(part 1 of 2)
# Autodesk Inventor assembly: Zynq_Z010_uZed_F_Prod
Saved by Autodesk Inventor 2015 (Build 190159000, 159)
## iProperties
Created: 2015-04-03
Part Number: Zynq_Z010_uZed_F_Prod
Document SubType Name: Assembly
Designer: -
Author: -
Author: Author
Title: Open CASCADE Shape Model
Organization: Open CASCADE
Description: Open CASCADE Model
Authority: Unknown
Creation Date: 2013-12-20
Sending System: Open CASCADE 6.2
Preprocessor: Open CASCADE STEP processor 6.2
## Documents named in this file (361)
- C:\Users\spichelh\Documents\GitHub\beta-hardware\Enclosure\Version 002\Imported Components\Zynq_Z010_uZed_F_Prod\Zynq_Z010_uZed_F_Prod.iam
- C:\Users\spichelh\Documents\GitHub\beta-hardware\Enclosure\Version 002\Imported Components\Zynq_Z010_uZed_F_Prod\Board.ipt
- C:\Users\spichelh\Documents\GitHub\beta-hardware\Enclosure\Version 002\Imported Components\Zynq_Z010_uZed_F_Prod\R96.iam
- C:\Users\spichelh\Documents\GitHub\beta-hardware\Enclosure\Version 002\Imported Components\Zynq_Z010_uZed_F_Prod\C220.iam
- C:\Users\spichelh\Documents\GitHub\beta-hardware\Enclosure\Version 002\Imported Components\Zynq_Z010_uZed_F_Prod\C219.iam
- C:\Users\spichelh\Documents\GitHub\beta-hardware\Enclosure\Version 002\Imported Components\Zynq_Z010_uZed_F_Prod\R91.iam
- C:\Users\spichelh\Documents\GitHub\beta-hardware\Enclosure\Version 002\Imported Components\Zynq_Z010_uZed_F_Prod\R90.iam
- C:\Users\spichelh\Documents\GitHub\beta-hardware\Enclosure\Version 002\Imported Components\Zynq_Z010_uZed_F_Prod\R89.iam
- C:\Users\spichelh\Documents\GitHub\beta-hardware\Enclosure\Version 002\Imported Components\Zynq_Z010_uZed_F_Prod\R88.iam
- C:\Users\spichelh\Documents\GitHub\beta-hardware\Enclosure\Version 002\Imported Components\Zynq_Z010_uZed_F_Prod\D1.iam
- C:\Users\spichelh\Documents\GitHub\beta-hardware\Enclosure\Version 002\Imported Components\Zynq_Z010_uZed_F_Prod\MTG3.iam
- C:\Users\spichelh\Documents\GitHub\beta-hardware\Enclosure\Version 002\Imported Components\Zynq_Z010_uZed_F_Prod\MTG4.iam
- C:\Users\spichelh\Documents\GitHub\beta-hardware\Enclosure\Version 002\Imported Components\Zynq_Z010_uZed_F_Prod\U11.iam
- C:\Users\spichelh\Documents\GitHub\beta-hardware\Enclosure\Version 002\Imported Components\Zynq_Z010_uZed_F_Prod\U5.iam
- C:\Users\spichelh\Documents\GitHub\beta-hardware\Enclosure\Version 002\Imported Components\Zynq_Z010_uZed_F_Prod\U6.iam
- C:\Users\spichelh\Documents\GitHub\beta-hardware\Enclosure\Version 002\Imported Components\Zynq_Z010_uZed_F_Prod\U10.iam
- C:\Users\spichelh\Documents\GitHub\beta-hardware\Enclosure\Version 002\Imported Components\Zynq_Z010_uZed_F_Prod\U13.iam
- C:\Users\spichelh\Documents\GitHub\beta-hardware\Enclosure\Version 002\Imported Components\Zynq_Z010_uZed_F_Prod\C41.iam
- C:\Users\spichelh\Documents\GitHub\beta-hardware\Enclosure\Version 002\Imported Components\Zynq_Z010_uZed_F_Prod\C170.iam
- C:\Users\spichelh\Documents\GitHub\beta-hardware\Enclosure\Version 002\Imported Components\Zynq_Z010_uZed_F_Prod\C176.iam
- C:\Users\spichelh\Documents\GitHub\beta-hardware\Enclosure\Version 002\Imported Components\Zynq_Z010_uZed_F_Prod\C181.iam
- C:\Users\spichelh\Documents\GitHub\beta-hardware\Enclosure\Version 002\Imported Components\Zynq_Z010_uZed_F_Prod\C188.iam
- C:\Users\spichelh\Documents\GitHub\beta-hardware\Enclosure\Version 002\Imported Components\Zynq_Z010_uZed_F_Prod\C42.iam
- C:\Users\spichelh\Documents\GitHub\beta-hardware\Enclosure\Version 002\Imported Components\Zynq_Z010_uZed_F_Prod\C190.iam
- C:\Users\spichelh\Documents\GitHub\beta-hardware\Enclosure\Version 002\Imported Components\Zynq_Z010_uZed_F_Prod\C179.iam
- C:\Users\spichelh\Documents\GitHub\beta-hardware\Enclosure\Version 002\Imported Components\Zynq_Z010_uZed_F_Prod\C189.iam
- C:\Users\spichelh\Documents\GitHub\beta-hardware\Enclosure\Version 002\Imported Components\Zynq_Z010_uZed_F_Prod\C169.iam
- C:\Users\spichelh\Documents\GitHub\beta-hardware\Enclosure\Version 002\Imported Components\Zynq_Z010_uZed_F_Prod\C193.iam
- C:\Users\spichelh\Documents\GitHub\beta-hardware\Enclosure\Version 002\Imported Components\Zynq_Z010_uZed_F_Prod\C196.iam
- C:\Users\spichelh\Documents\GitHub\beta-hardware\Enclosure\Version 002\Imported Components\Zynq_Z010_uZed_F_Prod\C200.iam
- C:\Users\spichelh\Documents\GitHub\beta-hardware\Enclosure\Version 002\Imported Components\Zynq_Z010_uZed_F_Prod\C203.iam
- C:\Users\spichelh\Documents\GitHub\beta-hardware\Enclosure\Version 002\Imported Components\Zynq_Z010_uZed_F_Prod\C173.iam
- C:\Users\spichelh\Documents\GitHub\beta-hardware\Enclosure\Version 002\Imported Components\Zynq_Z010_uZed_F_Prod\C175.iam
- C:\Users\spichelh\Documents\GitHub\beta-hardware\Enclosure\Version 002\Imported Components\Zynq_Z010_uZed_F_Prod\C171.iam
- C:\Users\spichelh\Documents\GitHub\beta-hardware\Enclosure\Version 002\Imported Components\Zynq_Z010_uZed_F_Prod\C183.iam
- C:\Users\spichelh\Documents\GitHub\beta-hardware\Enclosure\Version 002\Imported Components\Zynq_Z010_uZed_F_Prod\C43.iam
- C:\Users\spichelh\Documents\GitHub\beta-hardware\Enclosure\Version 002\Imported Components\Zynq_Z010_uZed_F_Prod\C199.iam
- C:\Users\spichelh\Documents\GitHub\beta-hardware\Enclosure\Version 002\Imported Components\Zynq_Z010_uZed_F_Prod\C194.iam
- C:\Users\spichelh\Documents\GitHub\beta-hardware\Enclosure\Version 002\Imported Components\Zynq_Z010_uZed_F_Prod\C186.iam
- C:\Users\spichelh\Documents\GitHub\beta-hardware\Enclosure\Version 002\Imported Components\Zynq_Z010_uZed_F_Prod\C184.iam
- C:\Users\spichelh\Documents\GitHub\beta-hardware\Enclosure\Version 002\Imported Components\Zynq_Z010_uZed_F_Prod\C44.iam
- C:\Users\spichelh\Documents\GitHub\beta-hardware\Enclosure\Version 002\Imported Components\Zynq_Z010_uZed_F_Prod\C202.iam
- C:\Users\spichelh\Documents\GitHub\beta-hardware\Enclosure\Version 002\Imported Components\Zynq_Z010_uZed_F_Prod\C201.iam
- C:\Users\spichelh\Documents\GitHub\beta-hardware\Enclosure\Version 002\Imported Components\Zynq_Z010_uZed_F_Prod\C182.iam
- C:\Users\spichelh\Documents\GitHub\beta-hardware\Enclosure\Version 002\Imported Components\Zynq_Z010_uZed_F_Prod\C177.iam
- C:\Users\spichelh\Documents\GitHub\beta-hardware\Enclosure\Version 002\Imported Components\Zynq_Z010_uZed_F_Prod\C180.iam
- C:\Users\spichelh\Documents\GitHub\beta-hardware\Enclosure\Version 002\Imported Components\Zynq_Z010_uZed_F_Prod\C178.iam
- C:\Users\spichelh\Documents\GitHub\beta-hardware\Enclosure\Version 002\Imported Components\Zynq_Z010_uZed_F_Prod\C172.iam
- C:\Users\spichelh\Documents\GitHub\beta-hardware\Enclosure\Version 002\Imported Components\Zynq_Z010_uZed_F_Prod\C174.iam
- C:\Users\spichelh\Documents\GitHub\beta-hardware\Enclosure\Version 002\Imported Components\Zynq_Z010_uZed_F_Prod\C197.iam
- C:\Users\spichelh\Documents\GitHub\beta-hardware\Enclosure\Version 002\Imported Components\Zynq_Z010_uZed_F_Prod\C192.iam
- C:\Users\spichelh\Documents\GitHub\beta-hardware\Enclosure\Version 002\Imported Components\Zynq_Z010_uZed_F_Prod\C198.iam
- C:\Users\spichelh\Documents\GitHub\beta-hardware\Enclosure\Version 002\Imported Components\Zynq_Z010_uZed_F_Prod\C191.iam
- C:\Users\spichelh\Documents\GitHub\beta-hardware\Enclosure\Version 002\Imported Components\Zynq_Z010_uZed_F_Prod\C187.iam
- C:\Users\spichelh\Documents\GitHub\beta-hardware\Enclosure\Version 002\Imported Components\Zynq_Z010_uZed_F_Prod\C148.iam
- C:\Users\spichelh\Documents\GitHub\beta-hardware\Enclosure\Version 002\Imported Components\Zynq_Z010_uZed_F_Prod\C195.iam
- C:\Users\spichelh\Documents\GitHub\beta-hardware\Enclosure\Version 002\Imported Components\Zynq_Z010_uZed_F_Prod\C149.iam
- C:\Users\spichelh\Documents\GitHub\beta-hardware\Enclosure\Version 002\Imported Components\Zynq_Z010_uZed_F_Prod\C205.iam
- C:\Users\spichelh\Documents\GitHub\beta-hardware\Enclosure\Version 002\Imported Components\Zynq_Z010_uZed_F_Prod\C48.iam
- C:\Users\spichelh\Documents\GitHub\beta-hardware\Enclosure\Version 002\Imported Components\Zynq_Z010_uZed_F_Prod\C55.iam
- C:\Users\spichelh\Documents\GitHub\beta-hardware\Enclosure\Version 002\Imported Components\Zynq_Z010_uZed_F_Prod\C49.iam
- C:\Users\spichelh\Documents\GitHub\beta-hardware\Enclosure\Version 002\Imported Components\Zynq_Z010_uZed_F_Prod\C47.iam
- C:\Users\spichelh\Documents\GitHub\beta-hardware\Enclosure\Version 002\Imported Components\Zynq_Z010_uZed_F_Prod\C46.iam
- C:\Users\spichelh\Documents\GitHub\beta-hardware\Enclosure\Version 002\Imported Components\Zynq_Z010_uZed_F_Prod\C39.iam
- C:\Users\spichelh\Documents\GitHub\beta-hardware\Enclosure\Version 002\Imported Components\Zynq_Z010_uZed_F_Prod\C45.iam
- C:\Users\spichelh\Documents\GitHub\beta-hardware\Enclosure\Version 002\Imported Components\Zynq_Z010_uZed_F_Prod\C185.iam
- C:\Users\spichelh\Documents\GitHub\beta-hardware\Enclosure\Version 002\Imported Components\Zynq_Z010_uZed_F_Prod\C204.iam
- C:\Users\spichelh\Documents\GitHub\beta-hardware\Enclosure\Version 002\Imported Components\Zynq_Z010_uZed_F_Prod\C37.iam
- C:\Users\spichelh\Documents\GitHub\beta-hardware\Enclosure\Version 002\Imported Components\Zynq_Z010_uZed_F_Prod\C38.iam
- C:\Users\spichelh\Documents\GitHub\beta-hardware\Enclosure\Version 002\Imported Components\Zynq_Z010_uZed_F_Prod\C7.iam
- C:\Users\spichelh\Documents\GitHub\beta-hardware\Enclosure\Version 002\Imported Components\Zynq_Z010_uZed_F_Prod\C8.iam
- C:\Users\spichelh\Documents\GitHub\beta-hardware\Enclosure\Version 002\Imported Components\Zynq_Z010_uZed_F_Prod\C5.iam
- C:\Users\spichelh\Documents\GitHub\beta-hardware\Enclosure\Version 002\Imported Components\Zynq_Z010_uZed_F_Prod\C2.iam
- C:\Users\spichelh\Documents\GitHub\beta-hardware\Enclosure\Version 002\Imported Components\Zynq_Z010_uZed_F_Prod\C93.iam
- C:\Users\spichelh\Documents\GitHub\beta-hardware\Enclosure\Version 002\Imported Components\Zynq_Z010_uZed_F_Prod\C73.iam
- C:\Users\spichelh\Documents\GitHub\beta-hardware\Enclosure\Version 002\Imported Components\Zynq_Z010_uZed_F_Prod\C87.iam
- C:\Users\spichelh\Documents\GitHub\beta-hardware\Enclosure\Version 002\Imported Components\Zynq_Z010_uZed_F_Prod\C74.iam
- C:\Users\spichelh\Documents\GitHub\beta-hardware\Enclosure\Version 002\Imported Components\Zynq_Z010_uZed_F_Prod\C90.iam
- C:\Users\spichelh\Documents\GitHub\beta-hardware\Enclosure\Version 002\Imported Components\Zynq_Z010_uZed_F_Prod\C78.iam
- C:\Users\spichelh\Documents\GitHub\beta-hardware\Enclosure\Version 002\Imported Components\Zynq_Z010_uZed_F_Prod\C86.iam
- C:\Users\spichelh\Documents\GitHub\beta-hardware\Enclosure\Version 002\Imported Components\Zynq_Z010_uZed_F_Prod\C88.iam
- C:\Users\spichelh\Documents\GitHub\beta-hardware\Enclosure\Version 002\Imported Components\Zynq_Z010_uZed_F_Prod\C81.iam
- C:\Users\spichelh\Documents\GitHub\beta-hardware\Enclosure\Version 002\Imported Components\Zynq_Z010_uZed_F_Prod\C85.iam
- C:\Users\spichelh\Documents\GitHub\beta-hardware\Enclosure\Version 002\Imported Components\Zynq_Z010_uZed_F_Prod\C11.iam
- C:\Users\spichelh\Documents\GitHub\beta-hardware\Enclosure\Version 002\Imported Components\Zynq_Z010_uZed_F_Prod\C83.iam
- C:\Users\spichelh\Documents\GitHub\beta-hardware\Enclosure\Version 002\Imported Components\Zynq_Z010_uZed_F_Prod\C79.iam
- C:\Users\spichelh\Documents\GitHub\beta-hardware\Enclosure\Version 002\Imported Components\Zynq_Z010_uZed_F_Prod\C75.iam
- C:\Users\spichelh\Documents\GitHub\beta-hardware\Enclosure\Version 002\Imported Components\Zynq_Z010_uZed_F_Prod\C92.iam
- C:\Users\spichelh\Documents\GitHub\beta-hardware\Enclosure\Version 002\Imported Components\Zynq_Z010_uZed_F_Prod\C12.iam
- C:\Users\spichelh\Documents\GitHub\beta-hardware\Enclosure\Version 002\Imported Components\Zynq_Z010_uZed_F_Prod\C80.iam
- C:\Users\spichelh\Documents\GitHub\beta-hardware\Enclosure\Version 002\Imported Components\Zynq_Z010_uZed_F_Prod\C82.iam
- C:\Users\spichelh\Documents\GitHub\beta-hardware\Enclosure\Version 002\Imported Components\Zynq_Z010_uZed_F_Prod\C84.iam
- C:\Users\spichelh\Documents\GitHub\beta-hardware\Enclosure\Version 002\Imported Components\Zynq_Z010_uZed_F_Prod\C10.iam
- C:\Users\spichelh\Documents\GitHub\beta-hardware\Enclosure\Version 002\Imported Components\Zynq_Z010_uZed_F_Prod\C1.iam
- C:\Users\spichelh\Documents\GitHub\beta-hardware\Enclosure\Version 002\Imported Components\Zynq_Z010_uZed_F_Prod\C68.iam
- C:\Users\spichelh\Documents\GitHub\beta-hardware\Enclosure\Version 002\Imported Components\Zynq_Z010_uZed_F_Prod\C67.iam
- C:\Users\spichelh\Documents\GitHub\beta-hardware\Enclosure\Version 002\Imported Components\Zynq_Z010_uZed_F_Prod\C76.iam
- C:\Users\spichelh\Documents\GitHub\beta-hardware\Enclosure\Version 002\Imported Components\Zynq_Z010_uZed_F_Prod\C9.iam
- C:\Users\spichelh\Documents\GitHub\beta-hardware\Enclosure\Version 002\Imported Components\Zynq_Z010_uZed_F_Prod\C72.iam
- C:\Users\spichelh\Documents\GitHub\beta-hardware\Enclosure\Version 002\Imported Components\Zynq_Z010_uZed_F_Prod\C71.iam
- C:\Users\spichelh\Documents\GitHub\beta-hardware\Enclosure\Version 002\Imported Components\Zynq_Z010_uZed_F_Prod\C77.iam
- C:\Users\spichelh\Documents\GitHub\beta-hardware\Enclosure\Version 002\Imported Components\Zynq_Z010_uZed_F_Prod\C62.iam
- C:\Users\spichelh\Documents\GitHub\beta-hardware\Enclosure\Version 002\Imported Components\Zynq_Z010_uZed_F_Prod\C209.iam
- C:\Users\spichelh\Documents\GitHub\beta-hardware\Enclosure\Version 002\Imported Components\Zynq_Z010_uZed_F_Prod\C206.iam
- C:\Users\spichelh\Documents\GitHub\beta-hardware\Enclosure\Version 002\Imported Components\Zynq_Z010_uZed_F_Prod\C32.iam
- C:\Users\spichelh\Documents\GitHub\beta-hardware\Enclosure\Version 002\Imported Components\Zynq_Z010_uZed_F_Prod\C34.iam
- C:\Users\spichelh\Documents\GitHub\beta-hardware\Enclosure\Version 002\Imported Components\Zynq_Z010_uZed_F_Prod\C35.iam
- C:\Users\spichelh\Documents\GitHub\beta-hardware\Enclosure\Version 002\Imported Components\Zynq_Z010_uZed_F_Prod\C207.iam
- C:\Users\spichelh\Documents\GitHub\beta-hardware\Enclosure\Version 002\Imported Components\Zynq_Z010_uZed_F_Prod\C215.iam
- C:\Users\spichelh\Documents\GitHub\beta-hardware\Enclosure\Version 002\Imported Components\Zynq_Z010_uZed_F_Prod\C216.iam
- C:\Users\spichelh\Documents\GitHub\beta-hardware\Enclosure\Version 002\Imported Components\Zynq_Z010_uZed_F_Prod\C33.iam
- C:\Users\spichelh\Documents\GitHub\beta-hardware\Enclosure\Version 002\Imported Components\Zynq_Z010_uZed_F_Prod\C36.iam
- C:\Users\spichelh\Documents\GitHub\beta-hardware\Enclosure\Version 002\Imported Components\Zynq_Z010_uZed_F_Prod\C31.iam
- C:\Users\spichelh\Documents\GitHub\beta-hardware\Enclosure\Version 002\Imported Components\Zynq_Z010_uZed_F_Prod\C211.iam
- C:\Users\spichelh\Documents\GitHub\beta-hardware\Enclosure\Version 002\Imported Components\Zynq_Z010_uZed_F_Prod\C210.iam
- C:\Users\spichelh\Documents\GitHub\beta-hardware\Enclosure\Version 002\Imported Components\Zynq_Z010_uZed_F_Prod\C208.iam
- C:\Users\spichelh\Documents\GitHub\beta-hardware\Enclosure\Version 002\Imported Components\Zynq_Z010_uZed_F_Prod\C50.iam
- C:\Users\spichelh\Documents\GitHub\beta-hardware\Enclosure\Version 002\Imported Components\Zynq_Z010_uZed_F_Prod\C213.iam
- C:\Users\spichelh\Documents\GitHub\beta-hardware\Enclosure\Version 002\Imported Components\Zynq_Z010_uZed_F_Prod\C214.iam
- C:\Users\spichelh\Documents\GitHub\beta-hardware\Enclosure\Version 002\Imported Components\Zynq_Z010_uZed_F_Prod\C24.iam
- C:\Users\spichelh\Documents\GitHub\beta-hardware\Enclosure\Version 002\Imported Components\Zynq_Z010_uZed_F_Prod\C25.iam
- C:\Users\spichelh\Documents\GitHub\beta-hardware\Enclosure\Version 002\Imported Components\Zynq_Z010_uZed_F_Prod\C26.iam
- C:\Users\spichelh\Documents\GitHub\beta-hardware\Enclosure\Version 002\Imported Components\Zynq_Z010_uZed_F_Prod\C151.iam
- C:\Users\spichelh\Documents\GitHub\beta-hardware\Enclosure\Version 002\Imported Components\Zynq_Z010_uZed_F_Prod\C111.iam
- C:\Users\spichelh\Documents\GitHub\beta-hardware\Enclosure\Version 002\Imported Components\Zynq_Z010_uZed_F_Prod\C20.iam
- C:\Users\spichelh\Documents\GitHub\beta-hardware\Enclosure\Version 002\Imported Components\Zynq_Z010_uZed_F_Prod\C117.iam
- C:\Users\spichelh\Documents\GitHub\beta-hardware\Enclosure\Version 002\Imported Components\Zynq_Z010_uZed_F_Prod\C94.iam
- C:\Users\spichelh\Documents\GitHub\beta-hardware\Enclosure\Version 002\Imported Components\Zynq_Z010_uZed_F_Prod\C118.iam
- C:\Users\spichelh\Documents\GitHub\beta-hardware\Enclosure\Version 002\Imported Components\Zynq_Z010_uZed_F_Prod\C119.iam
- C:\Users\spichelh\Documents\GitHub\beta-hardware\Enclosure\Version 002\Imported Components\Zynq_Z010_uZed_F_Prod\C141.iam
- C:\Users\spichelh\Documents\GitHub\beta-hardware\Enclosure\Version 002\Imported Components\Zynq_Z010_uZed_F_Prod\C40.iam
- C:\Users\spichelh\Documents\GitHub\beta-hardware\Enclosure\Version 002\Imported Components\Zynq_Z010_uZed_F_Prod\C129.iam
- C:\Users\spichelh\Documents\GitHub\beta-hardware\Enclosure\Version 002\Imported Components\Zynq_Z010_uZed_F_Prod\C140.iam
- C:\Users\spichelh\Documents\GitHub\beta-hardware\Enclosure\Version 002\Imported Components\Zynq_Z010_uZed_F_Prod\C157.iam
- C:\Users\spichelh\Documents\GitHub\beta-hardware\Enclosure\Version 002\Imported Components\Zynq_Z010_uZed_F_Prod\C14.iam
- C:\Users\spichelh\Documents\GitHub\beta-hardware\Enclosure\Version 002\Imported Components\Zynq_Z010_uZed_F_Prod\C16.iam
- C:\Users\spichelh\Documents\GitHub\beta-hardware\Enclosure\Version 002\Imported Components\Zynq_Z010_uZed_F_Prod\C101.iam
- C:\Users\spichelh\Documents\GitHub\beta-hardware\Enclosure\Version 002\Imported Components\Zynq_Z010_uZed_F_Prod\C97.iam
- C:\Users\spichelh\Documents\GitHub\beta-hardware\Enclosure\Version 002\Imported Components\Zynq_Z010_uZed_F_Prod\C145.iam
- C:\Users\spichelh\Documents\GitHub\beta-hardware\Enclosure\Version 002\Imported Components\Zynq_Z010_uZed_F_Prod\C121.iam
- C:\Users\spichelh\Documents\GitHub\beta-hardware\Enclosure\Version 002\Imported Components\Zynq_Z010_uZed_F_Prod\C126.iam
- C:\Users\spichelh\Documents\GitHub\beta-hardware\Enclosure\Version 002\Imported Components\Zynq_Z010_uZed_F_Prod\C125.iam
- C:\Users\spichelh\Documents\GitHub\beta-hardware\Enclosure\Version 002\Imported Components\Zynq_Z010_uZed_F_Prod\C128.iam
- C:\Users\spichelh\Documents\GitHub\beta-hardware\Enclosure\Version 002\Imported Components\Zynq_Z010_uZed_F_Prod\C150.iam
- C:\Users\spichelh\Documents\GitHub\beta-hardware\Enclosure\Version 002\Imported Components\Zynq_Z010_uZed_F_Prod\C131.iam
- C:\Users\spichelh\Documents\GitHub\beta-hardware\Enclosure\Version 002\Imported Components\Zynq_Z010_uZed_F_Prod\C138.iam
- C:\Users\spichelh\Documents\GitHub\beta-hardware\Enclosure\Version 002\Imported Components\Zynq_Z010_uZed_F_Prod\C144.iam
- C:\Users\spichelh\Documents\GitHub\beta-hardware\Enclosure\Version 002\Imported Components\Zynq_Z010_uZed_F_Prod\C147.iam
- C:\Users\spichelh\Documents\GitHub\beta-hardware\Enclosure\Version 002\Imported Components\Zynq_Z010_uZed_F_Prod\C154.iam
- C:\Users\spichelh\Documents\GitHub\beta-hardware\Enclosure\Version 002\Imported Components\Zynq_Z010_uZed_F_Prod\C103.iam
- C:\Users\spichelh\Documents\GitHub\beta-hardware\Enclosure\Version 002\Imported Components\Zynq_Z010_uZed_F_Prod\C102.iam
- C:\Users\spichelh\Documents\GitHub\beta-hardware\Enclosure\Version 002\Imported Components\Zynq_Z010_uZed_F_Prod\C100.iam
- C:\Users\spichelh\Documents\GitHub\beta-hardware\Enclosure\Version 002\Imported Components\Zynq_Z010_uZed_F_Prod\C99.iam
- C:\Users\spichelh\Documents\GitHub\beta-hardware\Enclosure\Version 002\Imported Components\Zynq_Z010_uZed_F_Prod\C98.iam
- C:\Users\spichelh\Documents\GitHub\beta-hardware\Enclosure\Version 002\Imported Components\Zynq_Z010_uZed_F_Prod\C13.iam
- C:\Users\spichelh\Documents\GitHub\beta-hardware\Enclosure\Version 002\Imported Components\Zynq_Z010_uZed_F_Prod\C110.iam
- C:\Users\spichelh\Documents\GitHub\beta-hardware\Enclosure\Version 002\Imported Components\Zynq_Z010_uZed_F_Prod\C108.iam
- C:\Users\spichelh\Documents\GitHub\beta-hardware\Enclosure\Version 002\Imported Components\Zynq_Z010_uZed_F_Prod\C17.iam
- C:\Users\spichelh\Documents\GitHub\beta-hardware\Enclosure\Version 002\Imported Components\Zynq_Z010_uZed_F_Prod\C160.iam
- C:\Users\spichelh\Documents\GitHub\beta-hardware\Enclosure\Version 002\Imported Components\Zynq_Z010_uZed_F_Prod\C23.iam
- C:\Users\spichelh\Documents\GitHub\beta-hardware\Enclosure\Version 002\Imported Components\Zynq_Z010_uZed_F_Prod\C133.iam
- C:\Users\spichelh\Documents\GitHub\beta-hardware\Enclosure\Version 002\Imported Components\Zynq_Z010_uZed_F_Prod\C112.iam
- C:\Users\spichelh\Documents\GitHub\beta-hardware\Enclosure\Version 002\Imported Components\Zynq_Z010_uZed_F_Prod\C96.iam
- C:\Users\spichelh\Documents\GitHub\beta-hardware\Enclosure\Version 002\Imported Components\Zynq_Z010_uZed_F_Prod\C142.iam
- C:\Users\spichelh\Documents\GitHub\beta-hardware\Enclosure\Version 002\Imported Components\Zynq_Z010_uZed_F_Prod\C21.iam
- C:\Users\spichelh\Documents\GitHub\beta-hardware\Enclosure\Version 002\Imported Components\Zynq_Z010_uZed_F_Prod\C123.iam
- C:\Users\spichelh\Documents\GitHub\beta-hardware\Enclosure\Version 002\Imported Components\Zynq_Z010_uZed_F_Prod\C120.iam
- C:\Users\spichelh\Documents\GitHub\beta-hardware\Enclosure\Version 002\Imported Components\Zynq_Z010_uZed_F_Prod\C30.iam
- C:\Users\spichelh\Documents\GitHub\beta-hardware\Enclosure\Version 002\Imported Components\Zynq_Z010_uZed_F_Prod\C29.iam
- C:\Users\spichelh\Documents\GitHub\beta-hardware\Enclosure\Version 002\Imported Components\Zynq_Z010_uZed_F_Prod\C162.iam
- C:\Users\spichelh\Documents\GitHub\beta-hardware\Enclosure\Version 002\Imported Components\Zynq_Z010_uZed_F_Prod\C164.iam
- C:\Users\spichelh\Documents\GitHub\beta-hardware\Enclosure\Version 002\Imported Components\Zynq_Z010_uZed_F_Prod\C166.iam
- C:\Users\spichelh\Documents\GitHub\beta-hardware\Enclosure\Version 002\Imported Components\Zynq_Z010_uZed_F_Prod\C165.iam
- C:\Users\spichelh\Documents\GitHub\beta-hardware\Enclosure\Version 002\Imported Components\Zynq_Z010_uZed_F_Prod\C27.iam
- C:\Users\spichelh\Documents\GitHub\beta-hardware\Enclosure\Version 002\Imported Components\Zynq_Z010_uZed_F_Prod\C158.iam
- C:\Users\spichelh\Documents\GitHub\beta-hardware\Enclosure\Version 002\Imported Components\Zynq_Z010_uZed_F_Prod\C153.iam
- C:\Users\spichelh\Documents\GitHub\beta-hardware\Enclosure\Version 002\Imported Components\Zynq_Z010_uZed_F_Prod\C155.iam
- C:\Users\spichelh\Documents\GitHub\beta-hardware\Enclosure\Version 002\Imported Components\Zynq_Z010_uZed_F_Prod\C105.iam
- C:\Users\spichelh\Documents\GitHub\beta-hardware\Enclosure\Version 002\Imported Components\Zynq_Z010_uZed_F_Prod\C106.iam
- C:\Users\spichelh\Documents\GitHub\beta-hardware\Enclosure\Version 002\Imported Components\Zynq_Z010_uZed_F_Prod\C104.iam
- C:\Users\spichelh\Documents\GitHub\beta-hardware\Enclosure\Version 002\Imported Components\Zynq_Z010_uZed_F_Prod\C109.iam
- C:\Users\spichelh\Documents\GitHub\beta-hardware\Enclosure\Version 002\Imported Components\Zynq_Z010_uZed_F_Prod\C107.iam
- C:\Users\spichelh\Documents\GitHub\beta-hardware\Enclosure\Version 002\Imported Components\Zynq_Z010_uZed_F_Prod\C15.iam
- C:\Users\spichelh\Documents\GitHub\beta-hardware\Enclosure\Version 002\Imported Components\Zynq_Z010_uZed_F_Prod\C146.iam
- C:\Users\spichelh\Documents\GitHub\beta-hardware\Enclosure\Version 002\Imported Components\Zynq_Z010_uZed_F_Prod\C95.iam
- C:\Users\spichelh\Documents\GitHub\beta-hardware\Enclosure\Version 002\Imported Components\Zynq_Z010_uZed_F_Prod\C113.iam
- C:\Users\spichelh\Documents\GitHub\beta-hardware\Enclosure\Version 002\Imported Components\Zynq_Z010_uZed_F_Prod\C91.iam
- C:\Users\spichelh\Documents\GitHub\beta-hardware\Enclosure\Version 002\Imported Components\Zynq_Z010_uZed_F_Prod\C134.iam
- C:\Users\spichelh\Documents\GitHub\beta-hardware\Enclosure\Version 002\Imported Components\Zynq_Z010_uZed_F_Prod\C135.iam
- C:\Users\spichelh\Documents\GitHub\beta-hardware\Enclosure\Version 002\Imported Components\Zynq_Z010_uZed_F_Prod\C168.iam
- C:\Users\spichelh\Documents\GitHub\beta-hardware\Enclosure\Version 002\Imported Components\Zynq_Z010_uZed_F_Prod\C163.iam
- C:\Users\spichelh\Documents\GitHub\beta-hardware\Enclosure\Version 002\Imported Components\Zynq_Z010_uZed_F_Prod\C167.iam
- C:\Users\spichelh\Documents\GitHub\beta-hardware\Enclosure\Version 002\Imported Components\Zynq_Z010_uZed_F_Prod\C161.iam
- C:\Users\spichelh\Documents\GitHub\beta-hardware\Enclosure\Version 002\Imported Components\Zynq_Z010_uZed_F_Prod\C159.iam
- C:\Users\spichelh\Documents\GitHub\beta-hardware\Enclosure\Version 002\Imported Components\Zynq_Z010_uZed_F_Prod\C19.iam
- C:\Users\spichelh\Documents\GitHub\beta-hardware\Enclosure\Version 002\Imported Components\Zynq_Z010_uZed_F_Prod\C114.iam
- C:\Users\spichelh\Documents\GitHub\beta-hardware\Enclosure\Version 002\Imported Components\Zynq_Z010_uZed_F_Prod\C122.iam
- C:\Users\spichelh\Documents\GitHub\beta-hardware\Enclosure\Version 002\Imported Components\Zynq_Z010_uZed_F_Prod\C132.iam
- C:\Users\spichelh\Documents\GitHub\beta-hardware\Enclosure\Version 002\Imported Components\Zynq_Z010_uZed_F_Prod\C124.iam
- C:\Users\spichelh\Documents\GitHub\beta-hardware\Enclosure\Version 002\Imported Components\Zynq_Z010_uZed_F_Prod\C89.iam
- C:\Users\spichelh\Documents\GitHub\beta-hardware\Enclosure\Version 002\Imported Components\Zynq_Z010_uZed_F_Prod\C116.iam
- C:\Users\spichelh\Documents\GitHub\beta-hardware\Enclosure\Version 002\Imported Components\Zynq_Z010_uZed_F_Prod\C22.iam
- C:\Users\spichelh\Documents\GitHub\beta-hardware\Enclosure\Version 002\Imported Components\Zynq_Z010_uZed_F_Prod\C6.iam
- C:\Users\spichelh\Documents\GitHub\beta-hardware\Enclosure\Version 002\Imported Components\Zynq_Z010_uZed_F_Prod\C57.iam
- C:\Users\spichelh\Documents\GitHub\beta-hardware\Enclosure\Version 002\Imported Components\Zynq_Z010_uZed_F_Prod\C58.iam
- C:\Users\spichelh\Documents\GitHub\beta-hardware\Enclosure\Version 002\Imported Components\Zynq_Z010_uZed_F_Prod\C64.iam
- C:\Users\spichelh\Documents\GitHub\beta-hardware\Enclosure\Version 002\Imported Components\Zynq_Z010_uZed_F_Prod\C56.iam
- C:\Users\spichelh\Documents\GitHub\beta-hardware\Enclosure\Version 002\Imported Components\Zynq_Z010_uZed_F_Prod\C59.iam
- C:\Users\spichelh\Documents\GitHub\beta-hardware\Enclosure\Version 002\Imported Components\Zynq_Z010_uZed_F_Prod\C63.iam
- C:\Users\spichelh\Documents\GitHub\beta-hardware\Enclosure\Version 002\Imported Components\Zynq_Z010_uZed_F_Prod\C51.iam
- C:\Users\spichelh\Documents\GitHub\beta-hardware\Enclosure\Version 002\Imported Components\Zynq_Z010_uZed_F_Prod\C53.iam
- C:\Users\spichelh\Documents\GitHub\beta-hardware\Enclosure\Version 002\Imported Components\Zynq_Z010_uZed_F_Prod\C60.iam
- C:\Users\spichelh\Documents\GitHub\beta-hardware\Enclosure\Version 002\Imported Components\Zynq_Z010_uZed_F_Prod\C52.iam
- C:\Users\spichelh\Documents\GitHub\beta-hardware\Enclosure\Version 002\Imported Components\Zynq_Z010_uZed_F_Prod\C54.iam
- C:\Users\spichelh\Documents\GitHub\beta-hardware\Enclosure\Version 002\Imported Components\Zynq_Z010_uZed_F_Prod\C61.iam
- C:\Users\spichelh\Documents\GitHub\beta-hardware\Enclosure\Version 002\Imported Components\Zynq_Z010_uZed_F_Prod\C3.iam
- C:\Users\spichelh\Documents\GitHub\beta-hardware\Enclosure\Version 002\Imported Components\Zynq_Z010_uZed_F_Prod\C152.iam
- C:\Users\spichelh\Documents\GitHub\beta-hardware\Enclosure\Version 002\Imported Components\Zynq_Z010_uZed_F_Prod\C70.iam
- C:\Users\spichelh\Documents\GitHub\beta-hardware\Enclosure\Version 002\Imported Components\Zynq_Z010_uZed_F_Prod\D3.iam
- C:\Users\spichelh\Documents\GitHub\beta-hardware\Enclosure\Version 002\Imported Components\Zynq_Z010_uZed_F_Prod\D9.iam
- C:\Users\spichelh\Documents\GitHub\beta-hardware\Enclosure\Version 002\Imported Components\Zynq_Z010_uZed_F_Prod\D7.iam
- C:\Users\spichelh\Documents\GitHub\beta-hardware\Enclosure\Version 002\Imported Components\Zynq_Z010_uZed_F_Prod\D5.iam
- C:\Users\spichelh\Documents\GitHub\beta-hardware\Enclosure\Version 002\Imported Components\Zynq_Z010_uZed_F_Prod\D2.iam
- C:\Users\spichelh\Documents\GitHub\beta-hardware\Enclosure\Version 002\Imported Components\Zynq_Z010_uZed_F_Prod\D6.iam
- C:\Users\spichelh\Documents\GitHub\beta-hardware\Enclosure\Version 002\Imported Components\Zynq_Z010_uZed_F_Prod\D8.iam
- C:\Users\spichelh\Documents\GitHub\beta-hardware\Enclosure\Version 002\Imported Components\Zynq_Z010_uZed_F_Prod\D4.iam
- C:\Users\spichelh\Documents\GitHub\beta-hardware\Enclosure\Version 002\Imported Components\Zynq_Z010_uZed_F_Prod\J6.iam
- C:\Users\spichelh\Documents\GitHub\beta-hardware\Enclosure\Version 002\Imported Components\Zynq_Z010_uZed_F_Prod\J5.iam
- C:\Users\spichelh\Documents\GitHub\beta-hardware\Enclosure\Version 002\Imported Components\Zynq_Z010_uZed_F_Prod\J1.iam
- C:\Users\spichelh\Documents\GitHub\beta-hardware\Enclosure\Version 002\Imported Components\Zynq_Z010_uZed_F_Prod\J3.iam
- C:\Users\spichelh\Documents\GitHub\beta-hardware\Enclosure\Version 002\Imported Components\Zynq_Z010_uZed_F_Prod\JP1.iam
- C:\Users\spichelh\Documents\GitHub\beta-hardware\Enclosure\Version 002\Imported Components\Zynq_Z010_uZed_F_Prod\JP2.iam
- C:\Users\spichelh\Documents\GitHub\beta-hardware\Enclosure\Version 002\Imported Components\Zynq_Z010_uZed_F_Prod\JP3.iam
- C:\Users\spichelh\Documents\GitHub\beta-hardware\Enclosure\Version 002\Imported Components\Zynq_Z010_uZed_F_Prod\JX1.iam
- C:\Users\spichelh\Documents\GitHub\beta-hardware\Enclosure\Version 002\Imported Components\Zynq_Z010_uZed_F_Prod\JX2.iam
- C:\Users\spichelh\Documents\GitHub\beta-hardware\Enclosure\Version 002\Imported Components\Zynq_Z010_uZed_F_Prod\L2.iam
- C:\Users\spichelh\Documents\GitHub\beta-hardware\Enclosure\Version 002\Imported Components\Zynq_Z010_uZed_F_Prod\L1.iam
- C:\Users\spichelh\Documents\GitHub\beta-hardware\Enclosure\Version 002\Imported Components\Zynq_Z010_uZed_F_Prod\L3.iam
- C:\Users\spichelh\Documents\GitHub\beta-hardware\Enclosure\Version 002\Imported Components\Zynq_Z010_uZed_F_Prod\L4.iam
- C:\Users\spichelh\Documents\GitHub\beta-hardware\Enclosure\Version 002\Imported Components\Zynq_Z010_uZed_F_Prod\L5.iam
- C:\Users\spichelh\Documents\GitHub\beta-hardware\Enclosure\Version 002\Imported Components\Zynq_Z010_uZed_F_Prod\Q1.iam
- C:\Users\spichelh\Documents\GitHub\beta-hardware\Enclosure\Version 002\Imported Components\Zynq_Z010_uZed_F_Prod\R79.iam
- C:\Users\spichelh\Documents\GitHub\beta-hardware\Enclosure\Version 002\Imported Components\Zynq_Z010_uZed_F_Prod\R85.iam
- C:\Users\spichelh\Documents\GitHub\beta-hardware\Enclosure\Version 002\Imported Components\Zynq_Z010_uZed_F_Prod\R74.iam
- C:\Users\spichelh\Documents\GitHub\beta-hardware\Enclosure\Version 002\Imported Components\Zynq_Z010_uZed_F_Prod\R75.iam
- C:\Users\spichelh\Documents\GitHub\beta-hardware\Enclosure\Version 002\Imported Components\Zynq_Z010_uZed_F_Prod\R29.iam
- C:\Users\spichelh\Documents\GitHub\beta-hardware\Enclosure\Version 002\Imported Components\Zynq_Z010_uZed_F_Prod\R27.iam
- C:\Users\spichelh\Documents\GitHub\beta-hardware\Enclosure\Version 002\Imported Components\Zynq_Z010_uZed_F_Prod\R80.iam
- C:\Users\spichelh\Documents\GitHub\beta-hardware\Enclosure\Version 002\Imported Components\Zynq_Z010_uZed_F_Prod\R84.iam
- C:\Users\spichelh\Documents\GitHub\beta-hardware\Enclosure\Version 002\Imported Components\Zynq_Z010_uZed_F_Prod\R78.iam
- C:\Users\spichelh\Documents\GitHub\beta-hardware\Enclosure\Version 002\Imported Components\Zynq_Z010_uZed_F_Prod\R33.iam
- C:\Users\spichelh\Documents\GitHub\beta-hardware\Enclosure\Version 002\Imported Components\Zynq_Z010_uZed_F_Prod\R32.iam
- C:\Users\spichelh\Documents\GitHub\beta-hardware\Enclosure\Version 002\Imported Components\Zynq_Z010_uZed_F_Prod\R24.iam
- C:\Users\spichelh\Documents\GitHub\beta-hardware\Enclosure\Version 002\Imported Components\Zynq_Z010_uZed_F_Prod\R31.iam
- C:\Users\spichelh\Documents\GitHub\beta-hardware\Enclosure\Version 002\Imported Components\Zynq_Z010_uZed_F_Prod\R30.iam
- C:\Users\spichelh\Documents\GitHub\beta-hardware\Enclosure\Version 002\Imported Components\Zynq_Z010_uZed_F_Prod\R86.iam
- C:\Users\spichelh\Documents\GitHub\beta-hardware\Enclosure\Version 002\Imported Components\Zynq_Z010_uZed_F_Prod\R28.iam
- C:\Users\spichelh\Documents\GitHub\beta-hardware\Enclosure\Version 002\Imported Components\Zynq_Z010_uZed_F_Prod\R83.iam
- C:\Users\spichelh\Documents\GitHub\beta-hardware\Enclosure\Version 002\Imported Components\Zynq_Z010_uZed_F_Prod\R26.iam
- C:\Users\spichelh\Documents\GitHub\beta-hardware\Enclosure\Version 002\Imported Components\Zynq_Z010_uZed_F_Prod\R23.iam
- C:\Users\spichelh\Documents\GitHub\beta-hardware\Enclosure\Version 002\Imported Components\Zynq_Z010_uZed_F_Prod\R82.iam
- C:\Users\spichelh\Documents\GitHub\beta-hardware\Enclosure\Version 002\Imported Components\Zynq_Z010_uZed_F_Prod\R21.iam
- C:\Users\spichelh\Documents\GitHub\beta-hardware\Enclosure\Version 002\Imported Components\Zynq_Z010_uZed_F_Prod\R25.iam
- C:\Users\spichelh\Documents\GitHub\beta-hardware\Enclosure\Version 002\Imported Components\Zynq_Z010_uZed_F_Prod\R81.iam
- C:\Users\spichelh\Documents\GitHub\beta-hardware\Enclosure\Version 002\Imported Components\Zynq_Z010_uZed_F_Prod\R22.iam
- C:\Users\spichelh\Documents\GitHub\beta-hardware\Enclosure\Version 002\Imported Components\Zynq_Z010_uZed_F_Prod\R18.iam
- C:\Users\spichelh\Documents\GitHub\beta-hardware\Enclosure\Version 002\Imported Components\Zynq_Z010_uZed_F_Prod\R20.iam
- C:\Users\spichelh\Documents\GitHub\beta-hardware\Enclosure\Version 002\Imported Components\Zynq_Z010_uZed_F_Prod\R19.iam
- C:\Users\spichelh\Documents\GitHub\beta-hardware\Enclosure\Version 002\Imported Components\Zynq_Z010_uZed_F_Prod\R17.iam
- C:\Users\spichelh\Documents\GitHub\beta-hardware\Enclosure\Version 002\Imported Components\Zynq_Z010_uZed_F_Prod\R16.iam
- C:\Users\spichelh\Documents\GitHub\beta-hardware\Enclosure\Version 002\Imported Components\Zynq_Z010_uZed_F_Prod\R14.iam
- C:\Users\spichelh\Documents\GitHub\beta-hardware\Enclosure\Version 002\Imported Components\Zynq_Z010_uZed_F_Prod\R77.iam
- C:\Users\spichelh\Documents\GitHub\beta-hardware\Enclosure\Version 002\Imported Components\Zynq_Z010_uZed_F_Prod\R15.iam
- C:\Users\spichelh\Documents\GitHub\beta-hardware\Enclosure\Version 002\Imported Components\Zynq_Z010_uZed_F_Prod\R64.iam
- C:\Users\spichelh\Documents\GitHub\beta-hardware\Enclosure\Version 002\Imported Components\Zynq_Z010_uZed_F_Prod\R71.iam
- C:\Users\spichelh\Documents\GitHub\beta-hardware\Enclosure\Version 002\Imported Components\Zynq_Z010_uZed_F_Prod\R3.iam
- C:\Users\spichelh\Documents\GitHub\beta-hardware\Enclosure\Version 002\Imported Components\Zynq_Z010_uZed_F_Prod\R7.iam
- C:\Users\spichelh\Documents\GitHub\beta-hardware\Enclosure\Version 002\Imported Components\Zynq_Z010_uZed_F_Prod\R70.iam
- C:\Users\spichelh\Documents\GitHub\beta-hardware\Enclosure\Version 002\Imported Components\Zynq_Z010_uZed_F_Prod\R8.iam
- C:\Users\spichelh\Documents\GitHub\beta-hardware\Enclosure\Version 002\Imported Components\Zynq_Z010_uZed_F_Prod\R76.iam
- C:\Users\spichelh\Documents\GitHub\beta-hardware\Enclosure\Version 002\Imported Components\Zynq_Z010_uZed_F_Prod\R4.iam
- C:\Users\spichelh\Documents\GitHub\beta-hardware\Enclosure\Version 002\Imported Components\Zynq_Z010_uZed_F_Prod\R54.iam
- C:\Users\spichelh\Documents\GitHub\beta-hardware\Enclosure\Version 002\Imported Components\Zynq_Z010_uZed_F_Prod\R47.iam
- C:\Users\spichelh\Documents\GitHub\beta-hardware\Enclosure\Version 002\Imported Components\Zynq_Z010_uZed_F_Prod\R62.iam
- C:\Users\spichelh\Documents\GitHub\beta-hardware\Enclosure\Version 002\Imported Components\Zynq_Z010_uZed_F_Prod\R13.iam
- C:\Users\spichelh\Documents\GitHub\beta-hardware\Enclosure\Version 002\Imported Components\Zynq_Z010_uZed_F_Prod\R63.iam
- C:\Users\spichelh\Documents\GitHub\beta-hardware\Enclosure\Version 002\Imported Components\Zynq_Z010_uZed_F_Prod\R60.iam
- C:\Users\spichelh\Documents\GitHub\beta-hardware\Enclosure\Version 002\Imported Components\Zynq_Z010_uZed_F_Prod\R55.iam
- C:\Users\spichelh\Documents\GitHub\beta-hardware\Enclosure\Version 002\Imported Components\Zynq_Z010_uZed_F_Prod\R58.iam
- C:\Users\spichelh\Documents\GitHub\beta-hardware\Enclosure\Version 002\Imported Components\Zynq_Z010_uZed_F_Prod\R61.iam
- C:\Users\spichelh\Documents\GitHub\beta-hardware\Enclosure\Version 002\Imported Components\Zynq_Z010_uZed_F_Prod\R6.iam
- C:\Users\spichelh\Documents\GitHub\beta-hardware\Enclosure\Version 002\Imported Components\Zynq_Z010_uZed_F_Prod\R56.iam
- C:\Users\spichelh\Documents\GitHub\beta-hardware\Enclosure\Version 002\Imported Components\Zynq_Z010_uZed_F_Prod\R50.iam
- C:\Users\spichelh\Documents\GitHub\beta-hardware\Enclosure\Version 002\Imported Components\Zynq_Z010_uZed_F_Prod\R73.iam
- C:\Users\spichelh\Documents\GitHub\beta-hardware\Enclosure\Version 002\Imported Components\Zynq_Z010_uZed_F_Prod\R72.iam
- C:\Users\spichelh\Documents\GitHub\beta-hardware\Enclosure\Version 002\Imported Components\Zynq_Z010_uZed_F_Prod\R66.iam
- C:\Users\spichelh\Documents\GitHub\beta-hardware\Enclosure\Version 002\Imported Components\Zynq_Z010_uZed_F_Prod\R65.iam
- C:\Users\spichelh\Documents\GitHub\beta-hardware\Enclosure\Version 002\Imported Components\Zynq_Z010_uZed_F_Prod\R59.iam
- C:\Users\spichelh\Documents\GitHub\beta-hardware\Enclosure\Version 002\Imported Components\Zynq_Z010_uZed_F_Prod\R51.iam
- C:\Users\spichelh\Documents\GitHub\beta-hardware\Enclosure\Version 002\Imported Components\Zynq_Z010_uZed_F_Prod\R9.iam
- C:\Users\spichelh\Documents\GitHub\beta-hardware\Enclosure\Version 002\Imported Components\Zynq_Z010_uZed_F_Prod\R67.iam
- C:\Users\spichelh\Documents\GitHub\beta-hardware\Enclosure\Version 002\Imported Components\Zynq_Z010_uZed_F_Prod\R10.iam
- C:\Users\spichelh\Documents\GitHub\beta-hardware\Enclosure\Version 002\Imported Components\Zynq_Z010_uZed_F_Prod\R68.iam
- C:\Users\spichelh\Documents\GitHub\beta-hardware\Enclosure\Version 002\Imported Components\Zynq_Z010_uZed_F_Prod\R5.iam
- C:\Users\spichelh\Documents\GitHub\beta-hardware\Enclosure\Version 002\Imported Components\Zynq_Z010_uZed_F_Prod\R57.iam
- C:\Users\spichelh\Documents\GitHub\beta-hardware\Enclosure\Version 002\Imported Components\Zynq_Z010_uZed_F_Prod\R87.iam
- C:\Users\spichelh\Documents\GitHub\beta-hardware\Enclosure\Version 002\Imported Components\Zynq_Z010_uZed_F_Prod\R42.iam
- C:\Users\spichelh\Documents\GitHub\beta-hardware\Enclosure\Version 002\Imported Components\Zynq_Z010_uZed_F_Prod\R45.iam
- C:\Users\spichelh\Documents\GitHub\beta-hardware\Enclosure\Version 002\Imported Components\Zynq_Z010_uZed_F_Prod\R1.iam
- C:\Users\spichelh\Documents\GitHub\beta-hardware\Enclosure\Version 002\Imported Components\Zynq_Z010_uZed_F_Prod\R46.iam
- C:\Users\spichelh\Documents\GitHub\beta-hardware\Enclosure\Version 002\Imported Components\Zynq_Z010_uZed_F_Prod\R12.iam
- C:\Users\spichelh\Documents\GitHub\beta-hardware\Enclosure\Version 002\Imported Components\Zynq_Z010_uZed_F_Prod\R41.iam
- C:\Users\spichelh\Documents\GitHub\beta-hardware\Enclosure\Version 002\Imported Components\Zynq_Z010_uZed_F_Prod\R40.iam
- C:\Users\spichelh\Documents\GitHub\beta-hardware\Enclosure\Version 002\Imported Components\Zynq_Z010_uZed_F_Prod\R11.iam
- C:\Users\spichelh\Documents\GitHub\beta-hardware\Enclosure\Version 002\Imported Components\Zynq_Z010_uZed_F_Prod\R43.iam
- C:\Users\spichelh\Documents\GitHub\beta-hardware\Enclosure\Version 002\Imported Components\Zynq_Z010_uZed_F_Prod\R34.iam
- C:\Users\spichelh\Documents\GitHub\beta-hardware\Enclosure\Version 002\Imported Components\Zynq_Z010_uZed_F_Prod\R38.iam
- C:\Users\spichelh\Documents\GitHub\beta-hardware\Enclosure\Version 002\Imported Components\Zynq_Z010_uZed_F_Prod\R44.iam
- C:\Users\spichelh\Documents\GitHub\beta-hardware\Enclosure\Version 002\Imported Components\Zynq_Z010_uZed_F_Prod\R39.iam
- C:\Users\spichelh\Documents\GitHub\beta-hardware\Enclosure\Version 002\Imported Components\Zynq_Z010_uZed_F_Prod\R35.iam
- C:\Users\spichelh\Documents\GitHub\beta-hardware\Enclosure\Version 002\Imported Components\Zynq_Z010_uZed_F_Prod\R36.iam
- C:\Users\spichelh\Documents\GitHub\beta-hardware\Enclosure\Version 002\Imported Components\Zynq_Z010_uZed_F_Prod\R37.iam
- C:\Users\spichelh\Documents\GitHub\beta-hardware\Enclosure\Version 002\Imported Components\Zynq_Z010_uZed_F_Prod\R69.iam
- C:\Users\spichelh\Documents\GitHub\beta-hardware\Enclosure\Version 002\Imported Components\Zynq_Z010_uZed_F_Prod\RP1.iam
- C:\Users\spichelh\Documents\GitHub\beta-hardware\Enclosure\Version 002\Imported Components\Zynq_Z010_uZed_F_Prod\RP2.iam
- C:\Users\spichelh\Documents\GitHub\beta-hardware\Enclosure\Version 002\Imported Components\Zynq_Z010_uZed_F_Prod\SW1.iam
- C:\Users\spichelh\Documents\GitHub\beta-hardware\Enclosure\Version 002\Imported Components\Zynq_Z010_uZed_F_Prod\SW2.iam
- C:\Users\spichelh\Documents\GitHub\beta-hardware\Enclosure\Version 002\Imported Components\Zynq_Z010_uZed_F_Prod\U9.iam
- C:\Users\spichelh\Documents\GitHub\beta-hardware\Enclosure\Version 002\Imported Components\Zynq_Z010_uZed_F_Prod\U12.iam
- C:\Users\spichelh\Documents\GitHub\beta-hardware\Enclosure\Version 002\Imported Components\Zynq_Z010_uZed_F_Prod\U1.iam
- C:\Users\spichelh\Documents\GitHub\beta-hardware\Enclosure\Version 002\Imported Components\Zynq_Z010_uZed_F_Prod\U7.iam
- C:\Users\spichelh\Documents\GitHub\beta-hardware\Enclosure\Version 002\Imported Components\Zynq_Z010_uZed_F_Prod\U19.iam
- C:\Users\spichelh\Documents\GitHub\beta-hardware\Enclosure\Version 002\Imported Components\Zynq_Z010_uZed_F_Prod\U4.iam
- C:\Users\spichelh\Documents\GitHub\beta-hardware\Enclosure\Version 002\Imported Components\Zynq_Z010_uZed_F_Prod\U20.iam
- C:\Users\spichelh\Documents\GitHub\beta-hardware\Enclosure\Version 002\Imported Components\Zynq_Z010_uZed_F_Prod\U8.iam
- C:\Users\spichelh\Documents\GitHub\beta-hardware\Enclosure\Version 002\Imported Components\Zynq_Z010_uZed_F_Prod\U17.iam
- C:\Users\spichelh\Documents\GitHub\beta-hardware\Enclosure\Version 002\Imported Components\Zynq_Z010_uZed_F_Prod\U2.iam
- C:\Users\spichelh\Documents\GitHub\beta-hardware\Enclosure\Version 002\Imported Components\Zynq_Z010_uZed_F_Prod\U16.iam
- C:\Users\spichelh\Documents\GitHub\beta-hardware\Enclosure\Version 002\Imported Components\Zynq_Z010_uZed_F_Prod\U14.iam
- C:\Users\spichelh\Documents\GitHub\beta-hardware\Enclosure\Version 002\Imported Components\Zynq_Z010_uZed_F_Prod\U15.iam
- C:\Users\spichelh\Documents\GitHub\beta-hardware\Enclosure\Version 002\Imported Components\Zynq_Z010_uZed_F_Prod\J2.iam
- C:\Users\spichelh\Documents\GitHub\beta-hardware\Enclosure\Version 002\Imported Components\Zynq_Z010_uZed_F_Prod\L8.iam
- C:\Users\spichelh\Documents\GitHub\beta-hardware\Enclosure\Version 002\Imported Components\Zynq_Z010_uZed_F_Prod\L9.iam
- C:\Users\spichelh\Documents\GitHub\beta-hardware\Enclosure\Version 002\Imported Components\Zynq_Z010_uZed_F_Prod\L6.iam
- C:\Users\spichelh\Documents\GitHub\beta-hardware\Enclosure\Version 002\Imported Components\Zynq_Z010_uZed_F_Prod\L7.iam
- C:\Users\spichelh\Documents\GitHub\beta-hardware\Enclosure\Version 002\Imported Components\Zynq_Z010_uZed_F_Prod\U3.iam
- C:\Users\spichelh\Documents\GitHub\beta-hardware\Enclosure\Version 002\Imported Components\Zynq_Z010_uZed_F_Prod\MTG5.iam
- C:\Users\spichelh\Documents\GitHub\beta-hardware\Enclosure\Version 002\Imported Components\Zynq_Z010_uZed_F_Prod\MTG2.iam
- C:\Users\spichelh\Documents\GitHub\beta-hardware\Enclosure\Version 002\Imported Components\Zynq_Z010_uZed_F_Prod\MTG1.iam
- C:\Users\spichelh\Documents\GitHub\beta-hardware\Enclosure\Version 002\Imported Components\Zynq_Z010_uZed_F_Prod\MTG6.iam
- C:\Users\spichelh\Documents\GitHub\beta-hardware\Enclosure\Version 002\Imported Components\Zynq_Z010_uZed_F_Prod\R92.iam
- C:\Users\spichelh\Documents\GitHub\beta-hardware\Enclosure\Version 002\Imported Components\Zynq_Z010_uZed_F_Prod\R93.iam
- C:\Users\spichelh\Documents\GitHub\beta-hardware\Enclosure\Version 002\Imported Components\Zynq_Z010_uZed_F_Prod\R94.iam
- C:\Users\spichelh\Documents\GitHub\beta-hardware\Enclosure\Version 002\Imported Components\Zynq_Z010_uZed_F_Prod\R95.iam
- C:\Users\spichelh\Documents\GitHub\beta-hardware\Enclosure\Version 002\Imported Components\Zynq_Z010_uZed_F_Prod\Q2.iam
- C:\Users\spichelh\Documents\GitHub\beta-hardware\Enclosure\Version 002\Imported Components\Zynq_Z010_uZed_F_Prod\Q3.iam
- C:\Users\spichelh\Documents\GitHub\beta-hardware\Enclosure\Version 002\Imported Components\Zynq_Z010_uZed_F_Prod\Q4.iam
- C:\Users\spichelh\Documents\GitHub\beta-hardware\Enclosure\Version 002\Imported Components\Zynq_Z010_uZed_F_Prod\Q5.iam
- C:\Users\spichelh\Documents\GitHub\beta-hardware\Enclosure\Version 002\Imported Components\Zynq_Z010_uZed_F_Prod\C221.iam
- C:\Users\spichelh\Documents\GitHub\beta-hardware\Enclosure\Version 002\Imported Components\Zynq_Z010_uZed_F_Prod\D10.iam
- C:\Users\spichelh\Documents\GitHub\beta-hardware\Enclosure\Version 002\Imported Components\Zynq_Z010_uZed_F_Prod\D12.iam
## Components (360 placed, 360 different names)
1. 1
2. 8 [sub-assembly]
3. 14 [sub-assembly]
4. 20 [sub-assembly]
5. 24 [sub-assembly]
6. 28 [sub-assembly]
7. 32 [sub-assembly]
8. 36 [sub-assembly]
9. 48 [sub-assembly]
10. 51 [sub-assembly]
11. 53 [sub-assembly]
12. 58 [sub-assembly]
13. 63 [sub-assembly]
14. 68 [sub-assembly]
15. 71 [sub-assembly]
16. 76 [sub-assembly]
17. 82 [sub-assembly]
18. 86 [sub-assembly]
19. 90 [sub-assembly]
20. 94 [sub-assembly]
21. 98 [sub-assembly]
22. 102 [sub-assembly]
23. 107 [sub-assembly]
24. 111 [sub-assembly]
25. 115 [sub-assembly]
26. 119 [sub-assembly]
27. 123 [sub-assembly]
28. 127 [sub-assembly]
29. 131 [sub-assembly]
30. 135 [sub-assembly]
31. 139 [sub-assembly]
32. 143 [sub-assembly]
33. 147 [sub-assembly]
34. 151 [sub-assembly]
35. 155 [sub-assembly]
36. 159 [sub-assembly]
37. 163 [sub-assembly]
38. 167 [sub-assembly]
39. 171 [sub-assembly]
40. 175 [sub-assembly]
41. 179 [sub-assembly]
42. 183 [sub-assembly]
43. 187 [sub-assembly]
44. 191 [sub-assembly]
45. 195 [sub-assembly]
46. 199 [sub-assembly]
47. 203 [sub-assembly]
48. 207 [sub-assembly]
49. 211 [sub-assembly]
50. 215 [sub-assembly]
51. 219 [sub-assembly]
52. 223 [sub-assembly]
53. 227 [sub-assembly]
54. 231 [sub-assembly]
55. 235 [sub-assembly]
56. 239 [sub-assembly]
57. 243 [sub-assembly]
58. 248 [sub-assembly]
59. 252 [sub-assembly]
60. 258 [sub-assembly]
61. 264 [sub-assembly]
62. 268 [sub-assembly]
63. 272 [sub-assembly]
64. 276 [sub-assembly]
65. 280 [sub-assembly]
66. 284 [sub-assembly]
67. 288 [sub-assembly]
68. 292 [sub-assembly]
69. 296 [sub-assembly]
70. 300 [sub-assembly]
71. 304 [sub-assembly]
72. 308 [sub-assembly]
73. 312 [sub-assembly]
74. 317 [sub-assembly]
75. 321 [sub-assembly]
76. 325 [sub-assembly]
77. 329 [sub-assembly]
78. 333 [sub-assembly]
79. 337 [sub-assembly]
80. 341 [sub-assembly]
81. 345 [sub-assembly]
82. 349 [sub-assembly]
83. 353 [sub-assembly]
84. 357 [sub-assembly]
85. 361 [sub-assembly]
86. 365 [sub-assembly]
87. 369 [sub-assembly]
88. 373 [sub-assembly]
89. 377 [sub-assembly]
90. 381 [sub-assembly]
91. 385 [sub-assembly]
92. 389 [sub-assembly]
93. 393 [sub-assembly]
94. 397 [sub-assembly]
95. 401 [sub-assembly]
96. 405 [sub-assembly]
97. 409 [sub-assembly]
98. 413 [sub-assembly]
99. 417 [sub-assembly]
100. 421 [sub-assembly]
101. 425 [sub-assembly]
102. 429 [sub-assembly]
103. 433 [sub-assembly]
104. 439 [sub-assembly]
105. 443 [sub-assembly]
106. 447 [sub-assembly]
107. 451 [sub-assembly]
108. 455 [sub-assembly]
109. 459 [sub-assembly]
110. 463 [sub-assembly]
111. 467 [sub-assembly]
112. 471 [sub-assembly]
113. 475 [sub-assembly]
114. 479 [sub-assembly]
115. 483 [sub-assembly]
116. 487 [sub-assembly]
117. 491 [sub-assembly]
118. 495 [sub-assembly]
119. 499 [sub-assembly]
120. 503 [sub-assembly]
121. 507 [sub-assembly]
122. 511 [sub-assembly]
123. 515 [sub-assembly]
124. 519 [sub-assembly]
125. 523 [sub-assembly]
126. 527 [sub-assembly]
127. 531 [sub-assembly]
128. 535 [sub-assembly]
129. 539 [sub-assembly]
130. 543 [sub-assembly]
131. 547 [sub-assembly]
132. 551 [sub-assembly]
133. 555 [sub-assembly]
134. 559 [sub-assembly]
135. 563 [sub-assembly]
136. 567 [sub-assembly]
137. 571 [sub-assembly]
138. 575 [sub-assembly]
139. 579 [sub-assembly]
140. 583 [sub-assembly]
141. 587 [sub-assembly]
142. 591 [sub-assembly]
143. 595 [sub-assembly]
144. 599 [sub-assembly]
145. 603 [sub-assembly]
146. 607 [sub-assembly]
147. 611 [sub-assembly]
148. 615 [sub-assembly]
149. 619 [sub-assembly]
150. 623 [sub-assembly]
151. 627 [sub-assembly]
152. 631 [sub-assembly]
153. 635 [sub-assembly]
154. 639 [sub-assembly]
155. 643 [sub-assembly]
156. 647 [sub-assembly]
157. 651 [sub-assembly]
158. 655 [sub-assembly]
159. 659 [sub-assembly]
160. 663 [sub-assembly]
161. 667 [sub-assembly]
162. 671 [sub-assembly]
163. 675 [sub-assembly]
164. 679 [sub-assembly]
165. 683 [sub-assembly]
166. 687 [sub-assembly]
167. 691 [sub-assembly]
168. 695 [sub-assembly]
169. 699 [sub-assembly]
170. 703 [sub-assembly]
171. 707 [sub-assembly]
172. 711 [sub-assembly]
173. 715 [sub-assembly]
174. 719 [sub-assembly]
175. 723 [sub-assembly]
176. 727 [sub-assembly]
177. 731 [sub-assembly]
178. 735 [sub-assembly]
179. 739 [sub-assembly]
180. 743 [sub-assembly]
181. 747 [sub-assembly]
182. 751 [sub-assembly]
183. 755 [sub-assembly]
184. 759 [sub-assembly]
185. 763 [sub-assembly]
186. 767 [sub-assembly]
187. 771 [sub-assembly]
188. 775 [sub-assembly]
189. 779 [sub-assembly]
190. 783 [sub-assembly]
191. 787 [sub-assembly]
192. 791 [sub-assembly]
193. 795 [sub-assembly]
194. 799 [sub-assembly]
195. 803 [sub-assembly]
196. 807 [sub-assembly]
197. 811 [sub-assembly]
198. 815 [sub-assembly]
199. 819 [sub-assembly]
200. 823 [sub-assembly]
201. 827 [sub-assembly]
202. 831 [sub-assembly]
203. 835 [sub-assembly]
204. 841 [sub-assembly]
205. 845 [sub-assembly]
206. 849 [sub-assembly]
207. 853 [sub-assembly]
208. 857 [sub-assembly]